# Autodesk Inventor assembly: Placed tall owen cupboard
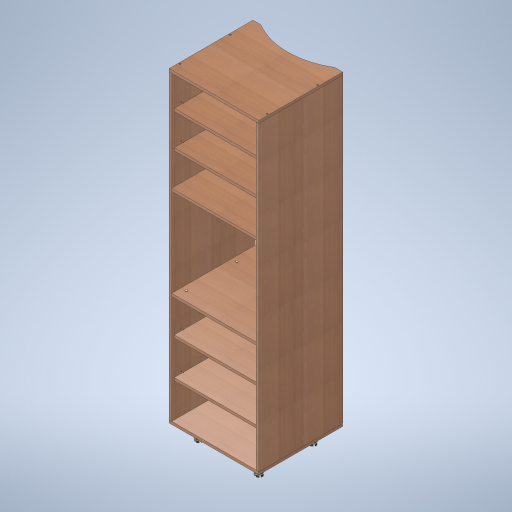
[picture p0: Inventor's stored thumbnail of the model, 512x512]
Saved by Autodesk Inventor 2024 (Build 280153000, 153)
## iProperties
RuleStatus: InUse
Created: 2017-02-07
Part Number: Placed tall owen cupboard
Document SubType Name: Assembly
Designer: SvetlanaB
Author: SvetlanaB
## Documents named in this file (23)
- C:\W4INV 2024 Design\iBOX LIBRARY\Kitchen\Standing Cabinets\Tall owen cupboard\Tall owen cupboard.iam
- C:\W4INV 2024 Design\iBOX LIBRARY\Kitchen\Standing Cabinets\Tall owen cupboard\Right panel.ipt
- C:\W4INV 2024 Design\iBOX LIBRARY\Kitchen\Standing Cabinets\Tall owen cupboard\Top panel.ipt
- C:\W4INV 2024 Design\iBOX LIBRARY\Kitchen\Standing Cabinets\Tall owen cupboard\Left panel.ipt
- C:\W4INV 2024 Design\iBOX LIBRARY\Kitchen\Standing Cabinets\Tall owen cupboard\Bottom panel.ipt
- C:\W4INV 2024 Design\iBOX LIBRARY\Kitchen\Standing Cabinets\Tall owen cupboard\Bottom shelf.ipt
- C:\W4INV 2024 Design\iBOX LIBRARY\Kitchen\Standing Cabinets\Tall owen cupboard\Bottom cupboard panel.ipt
- C:\W4INV 2024 Design\iBOX LIBRARY\Kitchen\Standing Cabinets\Tall owen cupboard\Top cupboard panel.ipt
- C:\W4INV 2024 Design\iBOX LIBRARY\Kitchen\Standing Cabinets\Tall owen cupboard\Top cupboard shelf.ipt
- C:\W4INV 2024 Design\iBOX LIBRARY\Kitchen\Standing Cabinets\Tall owen cupboard\Top cupboard back panel.ipt
- C:\W4INV 2024 Design\iBOX LIBRARY\Kitchen\Standing Cabinets\Tall owen cupboard\tall owen cupboard concept.ipt
- C:\W4INV 2024 Design\_LIBRARY\Holders\Shelf holder D5\Shelf support D5 L16 with hole covers.ipt
- C:\W4INV 2024 Design\_LIBRARY\Supports and legs\Legs\ADJUSTABLE LEG\Adjustable leg  BT18 clip included.ipt
- C:\W4INV 2024 Design\_LIBRARY\Supports and legs\Legs\ADJUSTABLE LEG\Adjustable leg  BT18.ipt
- C:\W4INV 2024 Design\_LIBRARY\Fixed joints\Confirmat\CONFIRMAT\Confirmat L50 NB T18 PB T 18.ipt
- C:\W4INV 2024 Design\_LIBRARY\Fixed joints\Minifix joint\MINIFIX D15 v2\Minifix D15 & Dowel L34 & Cap D15 PB T18 LH.ipt
- C:\W4INV 2024 Design\_LIBRARY\Fixed joints\Minifix joint\MINIFIX D15 v2\Minifix D15 & Dowel L34 & Cap D15 PB T18 RH.ipt
- C:\W4INV 2024 Design\iBOX LIBRARY\Kitchen\Standing Cabinets\Tall owen cupboard\Back.ipt
- C:\W4INV 2024 Design\_LIBRARY\Fixed joints\Confirmat\CONFIRMAT\Confirmat L50 & Cap D10 NB T18 PB T 18.ipt
- C:\W4INV 2023 Design\LIBRARY\Fixed joints\Confirmat\CONFIRMAT.ipt
- C:\W4INV 2023 Design\LIBRARY\Fixed joints\Minifix joint\MINIFIX D15 v2.ipt
- C:\W4INV 2023 Design\LIBRARY\Holders\Shelf holder D5.ipt
- C:\W4INV 2023 Design\LIBRARY\Supports and legs\Legs\ADJUSTABLE LEG.ipt
## Components (51 placed, 18 different names)
1. @Skeleton
2. Right panel:1 — Side Board Plane:3, Side Board Plane:4, Side Board Plane:7, Side Board Plane:8, Flush:11, Pillar Board Side Plane:1, Pillar Board Side Plane:3, Pillar Board Side Plane:6, Pillar Board Side Plane:8, Nestled Board Plane:6, Nestled Board Plane:12, Nestled Board Plane:14, Nestled Board Plane:16
3. Top panel:1 — Nestled Board Plane:1, Nestled Board Plane:2, Nestled Board Plane:3, Nestled Board Plane:4, Nestled Board Plane:18
4. Left panel:1 — Flush:1, Flush:2, Side Board Plane:1, Side Board Plane:2, Side Board Plane:5, Side Board Plane:6, Flush:12, Pillar Board Side Plane:2, Pillar Board Side Plane:4, Pillar Board Side Plane:5, Pillar Board Side Plane:7, Nestled Board Plane:5, Nestled Board Plane:11, Nestled Board Plane:13, Nestled Board Plane:15
5. Bottom panel:1 — Flush:13, Flush:14, Bottom board Plane:1, Front (Angle) Plane:1, Bottom board Plane:2, Front (Angle) Plane:2, Bottom board Plane:3, Front (Angle) Plane:3, Bottom board Plane:4, Front (Angle) Plane:4, Nestled Board Plane:7, Nestled Board Plane:8, Nestled Board Plane:9, Nestled Board Plane:10
6. Bottom cupboard panel:1 — Pillar Board Side Plane :1, Pillar Board Side Plane :2, Pillar Board Side Plane :5, Pillar Board Side Plane :6
7. Top cupboard panel:1 — Pillar Board Side Plane :3, Pillar Board Side Plane :4, Pillar Board Side Plane :7, Pillar Board Side Plane :8, Nestled Board Plane:17
8. Top cupboard back panel:1 — Pillar Board Side Plane :9, Pillar Board Side Plane :10
9. Back:1
10. Adjustable leg  BT18 clip included:1 — Axis2 Plane:1, Axis Plane:25, Bottom board Plane:1, Front (Angle) Plane:1
11. Adjustable leg  BT18 clip included:2 — Axis2 Plane:2, Axis Plane:26, Bottom board Plane:2, Front (Angle) Plane:2
12. Adjustable leg  BT18:3 — Axis2 Plane:3, Axis Plane:27, Bottom board Plane:3, Front (Angle) Plane:3
13. Adjustable leg  BT18:4 — Axis2 Plane:4, Axis Plane:28, Bottom board Plane:4, Front (Angle) Plane:4
14. Confirmat L50 & Cap D10 NB T18 PB T 18:1 — Axis Plane:1, Pillar Board Side Plane:1, Nestled Board Plane:1
15. Confirmat L50 & Cap D10 NB T18 PB T 18:2 — Axis Plane:2, Pillar Board Side Plane:2, Nestled Board Plane:2
16. Confirmat L50 & Cap D10 NB T18 PB T 18:3 — Axis Plane:3, Pillar Board Side Plane:3, Nestled Board Plane:3
17. Confirmat L50 & Cap D10 NB T18 PB T 18:4 — Axis Plane:4, Pillar Board Side Plane:4, Nestled Board Plane:4
18. Confirmat L50 NB T18 PB T 18:5 — Axis Plane:7, Pillar Board Side Plane:5, Nestled Board Plane:7
19. Confirmat L50 NB T18 PB T 18:6 — Axis Plane:8, Pillar Board Side Plane:6, Nestled Board Plane:8
20. Confirmat L50 NB T18 PB T 18:7 — Axis Plane:17, Pillar Board Side Plane:7, Nestled Board Plane:9
21. Confirmat L50 NB T18 PB T 18:8 — Axis Plane:18, Pillar Board Side Plane:8, Nestled Board Plane:10
22. Minifix D15 & Dowel L34 & Cap D15 PB T18 RH:1 — Axis Plane:5, Pillar Board Side Plane :1, Nestled Board Plane:5
23. Minifix D15 & Dowel L34 & Cap D15 PB T18 LH:2 — Axis Plane:6, Pillar Board Side Plane :2, Nestled Board Plane:6
24. Minifix D15 & Dowel L34 & Cap D15 PB T18 LH:3 — Axis Plane:19, Pillar Board Side Plane :3, Nestled Board Plane:11
25. Minifix D15 & Dowel L34 & Cap D15 PB T18 RH:4 — Axis Plane:20, Pillar Board Side Plane :4, Nestled Board Plane:12
26. Minifix D15 & Dowel L34 & Cap D15 PB T18 LH:5 — Axis Plane:21, Pillar Board Side Plane :5, Nestled Board Plane:13
27. Minifix D15 & Dowel L34 & Cap D15 PB T18 LH:6 — Axis Plane:22, Pillar Board Side Plane :6, Nestled Board Plane:14
28. Minifix D15 & Dowel L34 & Cap D15 PB T18 RH:7 — Axis Plane:23, Pillar Board Side Plane :7, Nestled Board Plane:15
29. Minifix D15 & Dowel L34 & Cap D15 PB T18 LH:8 — Axis Plane:24, Pillar Board Side Plane :8, Nestled Board Plane:16
30. Minifix D15 & Dowel L34 & Cap D15 PB T18 RH:9 — Nestled Board Plane:17, Pillar Board Side Plane :9, Axis Plane:29
31. Minifix D15 & Dowel L34 & Cap D15 PB T18 RH:10 — Nestled Board Plane:18, Pillar Board Side Plane :10, Axis Plane:30
32. Top cupboard shelf:1 — Shelf Pottom Plane:1, Shelf Pottom Plane:3, Shelf Pottom Plane:2, Shelf Pottom Plane:4
33. Shelf support D5 L16 with hole covers:2 — Axis Plane:9, Side Board Plane:1, Shelf Pottom Plane:1
34. Shelf support D5 L16 with hole covers:5 — Side Board Plane:2, Shelf Pottom Plane:2, Axis Plane:10
35. Shelf support D5 L16 with hole covers:4 — Axis Plane:11, Side Board Plane:3, Shelf Pottom Plane:3
36. Shelf support D5 L16 with hole covers:6 — Side Board Plane:4, Shelf Pottom Plane:4, Axis Plane:12
37. Top cupboard shelf:2
38. Shelf support D5 L16 with hole covers:23
39. Shelf support D5 L16 with hole covers:24
40. Shelf support D5 L16 with hole covers:25
41. Shelf support D5 L16 with hole covers:26
42. Bottom shelf:1 — Shelf Pottom Plane:5, Shelf Pottom Plane:6, Shelf Pottom Plane:7, Shelf Pottom Plane:8
43. Shelf support D5 L16 with hole covers:11 — Axis Plane:13, Side Board Plane:5, Shelf Pottom Plane:5
44. Shelf support D5 L16 with hole covers:12 — Axis Plane:14, Side Board Plane:6, Shelf Pottom Plane:6
45. Shelf support D5 L16 with hole covers:14 — Axis Plane:16, Side Board Plane:8, Shelf Pottom Plane:8
46. Shelf support D5 L16 with hole covers:13 — Axis Plane:15, Side Board Plane:7, Shelf Pottom Plane:7
47. Bottom shelf:2
48. Shelf support D5 L16 with hole covers:19
49. Shelf support D5 L16 with hole covers:20
50. Shelf support D5 L16 with hole covers:21
51. Shelf support D5 L16 with hole covers:22
## Component patterns: (2 elements, first: Top cupboard shelf:1 + Shelf support D5 L16 with hole covers:2 + Shelf support D5 L16 with hole covers:5 + Shelf support D5 L16 with hole covers:4 + Shelf support D5 L16 with hole covers:6), (2 elements, first: Bottom shelf:1 + Shelf support D5 L16 with hole covers:11 + Shelf support D5 L16 with hole covers:12 + Shelf support D5 L16 with hole covers:14 + Shelf support D5 L16 with hole covers:13)
## Relationships (100: Mate 72, Flush 24, Angle 4)
- Flush:1 (-64 mm): Left panel:1
- Flush:2 (-160 mm): Left panel:1
- Axis Plane:9 [Mate]: Shelf support D5 L16 with hole covers:2
- Side Board Plane:1 [Mate]: Left panel:1 ↔ Shelf support D5 L16 with hole covers:2
- Shelf Pottom Plane:1 [Mate] (2.5 mm): Top cupboard shelf:1 ↔ Shelf support D5 L16 with hole covers:2
- Axis Plane:11 [Mate]: Shelf support D5 L16 with hole covers:4
- Side Board Plane:3 [Mate]: Right panel:1 ↔ Shelf support D5 L16 with hole covers:4
- Shelf Pottom Plane:3 [Mate] (2.5 mm): Top cupboard shelf:1 ↔ Shelf support D5 L16 with hole covers:4
- Side Board Plane:2 [Mate]: Left panel:1 ↔ Shelf support D5 L16 with hole covers:5
- Shelf Pottom Plane:2 [Mate] (2.5 mm): Top cupboard shelf:1 ↔ Shelf support D5 L16 with hole covers:5
- Axis Plane:10 [Mate]: Shelf support D5 L16 with hole covers:5
- Side Board Plane:4 [Mate]: Right panel:1 ↔ Shelf support D5 L16 with hole covers:6
- Shelf Pottom Plane:4 [Mate] (2.5 mm): Top cupboard shelf:1 ↔ Shelf support D5 L16 with hole covers:6
- Axis Plane:12 [Mate]: Shelf support D5 L16 with hole covers:6
- Axis Plane:13 [Mate]: Shelf support D5 L16 with hole covers:11
- Side Board Plane:5 [Mate]: Left panel:1 ↔ Shelf support D5 L16 with hole covers:11
- Shelf Pottom Plane:5 [Mate] (2.5 mm): Bottom shelf:1 ↔ Shelf support D5 L16 with hole covers:11
- Axis Plane:14 [Mate]: Shelf support D5 L16 with hole covers:12
- Side Board Plane:6 [Mate]: Left panel:1 ↔ Shelf support D5 L16 with hole covers:12
- Shelf Pottom Plane:6 [Mate] (2.5 mm): Bottom shelf:1 ↔ Shelf support D5 L16 with hole covers:12
- Axis Plane:15 [Mate]: Shelf support D5 L16 with hole covers:13
- Side Board Plane:7 [Mate]: Right panel:1 ↔ Shelf support D5 L16 with hole covers:13
- Shelf Pottom Plane:7 [Mate] (2.5 mm): Bottom shelf:1 ↔ Shelf support D5 L16 with hole covers:13
- Axis Plane:16 [Mate]: Shelf support D5 L16 with hole covers:14
- Side Board Plane:8 [Mate]: Right panel:1 ↔ Shelf support D5 L16 with hole covers:14
- Shelf Pottom Plane:8 [Mate] (2.5 mm): Bottom shelf:1 ↔ Shelf support D5 L16 with hole covers:14
- Flush:11 (-100 mm): Right panel:1
- Flush:12 (-100 mm): Left panel:1
- Flush:13 (-100 mm): Bottom panel:1
- Flush:14 (-100 mm): Bottom panel:1
- Axis2 Plane:1 [Mate]: Adjustable leg  BT18 clip included:1
- Axis Plane:25 [Mate]: Adjustable leg  BT18 clip included:1
- Bottom board Plane:1 [Mate]: Bottom panel:1 ↔ Adjustable leg  BT18 clip included:1
- Front (Angle) Plane:1 [Angle] (0 deg): Bottom panel:1 ↔ Adjustable leg  BT18 clip included:1
- Axis2 Plane:2 [Mate]: Adjustable leg  BT18 clip included:2
- Axis Plane:26 [Mate]: Adjustable leg  BT18 clip included:2
- Bottom board Plane:2 [Mate]: Bottom panel:1 ↔ Adjustable leg  BT18 clip included:2
- Front (Angle) Plane:2 [Angle] (0 deg): Bottom panel:1 ↔ Adjustable leg  BT18 clip included:2
- Axis2 Plane:3 [Mate]: Adjustable leg  BT18:3
- Axis Plane:27 [Mate]: Adjustable leg  BT18:3
- Bottom board Plane:3 [Mate]: Bottom panel:1 ↔ Adjustable leg  BT18:3
- Front (Angle) Plane:3 [Angle] (0 deg): Bottom panel:1 ↔ Adjustable leg  BT18:3
- Axis2 Plane:4 [Mate]: Adjustable leg  BT18:4
- Axis Plane:28 [Mate]: Adjustable leg  BT18:4
- Bottom board Plane:4 [Mate]: Bottom panel:1 ↔ Adjustable leg  BT18:4
- Front (Angle) Plane:4 [Angle] (0 deg): Bottom panel:1 ↔ Adjustable leg  BT18:4
- Axis Plane:1 [Mate]: Confirmat L50 & Cap D10 NB T18 PB T 18:1
- Pillar Board Side Plane:1 [Mate] (-9 mm): Right panel:1 ↔ Confirmat L50 & Cap D10 NB T18 PB T 18:1
- Nestled Board Plane:1 [Flush]: Top panel:1 ↔ Confirmat L50 & Cap D10 NB T18 PB T 18:1
- Axis Plane:2 [Mate]: Confirmat L50 & Cap D10 NB T18 PB T 18:2
- Pillar Board Side Plane:2 [Mate] (-9 mm): Left panel:1 ↔ Confirmat L50 & Cap D10 NB T18 PB T 18:2
- Nestled Board Plane:2 [Flush]: Top panel:1 ↔ Confirmat L50 & Cap D10 NB T18 PB T 18:2
- Axis Plane:3 [Mate]: Confirmat L50 & Cap D10 NB T18 PB T 18:3
- Pillar Board Side Plane:3 [Mate] (-9 mm): Right panel:1 ↔ Confirmat L50 & Cap D10 NB T18 PB T 18:3
- Nestled Board Plane:3 [Flush]: Top panel:1 ↔ Confirmat L50 & Cap D10 NB T18 PB T 18:3
- Axis Plane:4 [Mate]: Confirmat L50 & Cap D10 NB T18 PB T 18:4
- Pillar Board Side Plane:4 [Mate] (-9 mm): Left panel:1 ↔ Confirmat L50 & Cap D10 NB T18 PB T 18:4
- Nestled Board Plane:4 [Flush]: Top panel:1 ↔ Confirmat L50 & Cap D10 NB T18 PB T 18:4
- Axis Plane:7 [Mate]: Confirmat L50 NB T18 PB T 18:5
- Pillar Board Side Plane:5 [Mate] (-9 mm): Left panel:1 ↔ Confirmat L50 NB T18 PB T 18:5
- Nestled Board Plane:7 [Flush]: Bottom panel:1 ↔ Confirmat L50 NB T18 PB T 18:5
- Axis Plane:8 [Mate]: Confirmat L50 NB T18 PB T 18:6
- Pillar Board Side Plane:6 [Mate] (-9 mm): Right panel:1 ↔ Confirmat L50 NB T18 PB T 18:6
- Nestled Board Plane:8 [Flush]: Bottom panel:1 ↔ Confirmat L50 NB T18 PB T 18:6
- Axis Plane:17 [Mate]: Confirmat L50 NB T18 PB T 18:7
- Pillar Board Side Plane:7 [Mate] (-9 mm): Left panel:1 ↔ Confirmat L50 NB T18 PB T 18:7
- Nestled Board Plane:9 [Flush]: Bottom panel:1 ↔ Confirmat L50 NB T18 PB T 18:7
- Axis Plane:18 [Mate]: Confirmat L50 NB T18 PB T 18:8
- Pillar Board Side Plane:8 [Mate] (-9 mm): Right panel:1 ↔ Confirmat L50 NB T18 PB T 18:8
- Nestled Board Plane:10 [Flush]: Bottom panel:1 ↔ Confirmat L50 NB T18 PB T 18:8
- Axis Plane:5 [Mate]: Minifix D15 & Dowel L34 & Cap D15 PB T18 RH:1
- Pillar Board Side Plane :1 [Flush] (18 mm): Bottom cupboard panel:1 ↔ Minifix D15 & Dowel L34 & Cap D15 PB T18 RH:1
- Nestled Board Plane:5 [Mate]: Left panel:1 ↔ Minifix D15 & Dowel L34 & Cap D15 PB T18 RH:1
- Axis Plane:6 [Mate]: Minifix D15 & Dowel L34 & Cap D15 PB T18 LH:2
- Pillar Board Side Plane :2 [Flush] (18 mm): Bottom cupboard panel:1 ↔ Minifix D15 & Dowel L34 & Cap D15 PB T18 LH:2
- Nestled Board Plane:6 [Mate]: Right panel:1 ↔ Minifix D15 & Dowel L34 & Cap D15 PB T18 LH:2
- Axis Plane:19 [Mate]: Minifix D15 & Dowel L34 & Cap D15 PB T18 LH:3
- Pillar Board Side Plane :3 [Flush] (18 mm): Top cupboard panel:1 ↔ Minifix D15 & Dowel L34 & Cap D15 PB T18 LH:3
- Nestled Board Plane:11 [Mate]: Left panel:1 ↔ Minifix D15 & Dowel L34 & Cap D15 PB T18 LH:3
- Axis Plane:20 [Mate]: Minifix D15 & Dowel L34 & Cap D15 PB T18 RH:4
- Pillar Board Side Plane :4 [Flush] (18 mm): Top cupboard panel:1 ↔ Minifix D15 & Dowel L34 & Cap D15 PB T18 RH:4
- Nestled Board Plane:12 [Mate]: Right panel:1 ↔ Minifix D15 & Dowel L34 & Cap D15 PB T18 RH:4
- Axis Plane:21 [Mate]: Minifix D15 & Dowel L34 & Cap D15 PB T18 LH:5
- Pillar Board Side Plane :5 [Flush] (18 mm): Bottom cupboard panel:1 ↔ Minifix D15 & Dowel L34 & Cap D15 PB T18 LH:5
- Nestled Board Plane:13 [Mate]: Left panel:1 ↔ Minifix D15 & Dowel L34 & Cap D15 PB T18 LH:5
- Axis Plane:22 [Mate]: Minifix D15 & Dowel L34 & Cap D15 PB T18 LH:6
- Pillar Board Side Plane :6 [Flush] (18 mm): Bottom cupboard panel:1 ↔ Minifix D15 & Dowel L34 & Cap D15 PB T18 LH:6
- Nestled Board Plane:14 [Mate]: Right panel:1 ↔ Minifix D15 & Dowel L34 & Cap D15 PB T18 LH:6
- Axis Plane:23 [Mate]: Minifix D15 & Dowel L34 & Cap D15 PB T18 RH:7
- Pillar Board Side Plane :7 [Flush] (18 mm): Top cupboard panel:1 ↔ Minifix D15 & Dowel L34 & Cap D15 PB T18 RH:7
- Nestled Board Plane:15 [Mate]: Left panel:1 ↔ Minifix D15 & Dowel L34 & Cap D15 PB T18 RH:7
- Axis Plane:24 [Mate]: Minifix D15 & Dowel L34 & Cap D15 PB T18 LH:8
- Pillar Board Side Plane :8 [Flush] (18 mm): Top cupboard panel:1 ↔ Minifix D15 & Dowel L34 & Cap D15 PB T18 LH:8
- Nestled Board Plane:16 [Mate]: Right panel:1 ↔ Minifix D15 & Dowel L34 & Cap D15 PB T18 LH:8
- Nestled Board Plane:17 [Mate]: Top cupboard panel:1 ↔ Minifix D15 & Dowel L34 & Cap D15 PB T18 RH:9
- Pillar Board Side Plane :9 [Flush] (18 mm): Top cupboard back panel:1 ↔ Minifix D15 & Dowel L34 & Cap D15 PB T18 RH:9
- Axis Plane:29 [Mate]: Minifix D15 & Dowel L34 & Cap D15 PB T18 RH:9
- Nestled Board Plane:18 [Mate]: Top panel:1 ↔ Minifix D15 & Dowel L34 & Cap D15 PB T18 RH:10
- Pillar Board Side Plane :10 [Flush] (18 mm): Top cupboard back panel:1 ↔ Minifix D15 & Dowel L34 & Cap D15 PB T18 RH:10
- Axis Plane:30 [Mate]: Minifix D15 & Dowel L34 & Cap D15 PB T18 RH:10
## Named parameters: Top_cupboard_shelf_quantity = 2, Bottom_shelf_quantity = 2, Panel_thickness = 18 mm, Place_for_owen = 590 mm, Owen_Place_from_Bottom = 750 mm, Distane_between_bottom_shelfs = 229 mm, Distance_between_top_shelfs = 209.66667 mm
